# Autodesk Inventor assembly: Y-Anchor
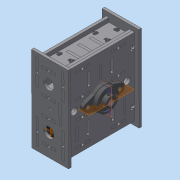
[picture p0: Inventor's stored thumbnail of the model, 180x180]
Saved by Autodesk Inventor 2016 SP1 (Build 200210100, 210)
## iProperties
Created: 2016-01-20
Part Number: Y-Anchor
Document SubType Name: Assembly
Designer: Mohamed A.
Author: Mohamed A.
## Documents named in this file (10)
- C:\Users\Mohamed\Documents\inventor\StemCellsPlatform\Laser Cut\Y-Anchor\Y-Anchor.iam
- C:\Users\Mohamed\Documents\inventor\StemCellsPlatform\Bearings\LM8UU 8mm Linear Bearing.ipt
- C:\Users\Mohamed\Documents\inventor\StemCellsPlatform\Laser Cut\Y-Anchor\Y-Anchor_Front-Outer.ipt
- C:\Users\Mohamed\Documents\inventor\StemCellsPlatform\Laser Cut\Y-Anchor\Y-Anchor_Front-Inner.ipt
- C:\Users\Mohamed\Documents\inventor\StemCellsPlatform\Laser Cut\Y-Anchor\Y-Anchor_Bearing-Ring-Middle.ipt
- C:\Users\Mohamed\Documents\inventor\StemCellsPlatform\Laser Cut\Y-Anchor\Y-Anchor_Bearing-Ring-Outer.ipt
- C:\Users\Mohamed\Documents\inventor\StemCellsPlatform\Laser Cut\Y-Anchor\X-Anchor_Bearing_Ring_Top.ipt
- C:\Users\Mohamed\Documents\inventor\StemCellsPlatform\Laser Cut\Y-Anchor\X-Anchor_Bearing_Ring_Top_Single.ipt
- C:\Users\Mohamed\Documents\inventor\StemCellsPlatform\Laser Cut\Y-Anchor\X-Anchor-Side.ipt
- C:\Users\Mohamed\Documents\inventor\StemCellsPlatform\Flanges\UFL08 -Housing.ipt
## Components (20 placed, 9 different names)
1. Y-Anchor_Front-Outer:1 — Mate:1, Mate:2, Mate:3
2. LM8UU 8mm Linear Bearing:1
3. LM8UU 8mm Linear Bearing:2
4. LM8UU 8mm Linear Bearing:4
5. Y-Anchor_Front-Inner:2
6. Y-Anchor_Bearing-Ring-Middle:2
7. Y-Anchor_Bearing-Ring-Middle:3
8. Y-Anchor_Bearing-Ring-Middle:4
9. Y-Anchor_Bearing-Ring-Outer:1
10. Y-Anchor_Front-Outer:2
11. X-Anchor_Bearing_Ring_Top_Single:2
12. Y-Anchor_Bearing-Ring-Outer:2
13. Y-Anchor_Bearing-Ring-Outer:3
14. Y-Anchor_Bearing-Ring-Outer:4
15. X-Anchor_Bearing_Ring_Top:2
16. X-Anchor_Bearing_Ring_Top_Single:1
17. X-Anchor_Bearing_Ring_Top:4
18. X-Anchor-Side:1
19. X-Anchor-Side:2
20. UFL08 -Housing:1 — Mate:1, Mate:2, Mate:3
## Relationships (3: Mate 3)
- Mate:1: Y-Anchor_Front-Outer:1 ↔ UFL08 -Housing:1
- Mate:2: Y-Anchor_Front-Outer:1 ↔ UFL08 -Housing:1
- Mate:3: Y-Anchor_Front-Outer:1 ↔ UFL08 -Housing:1
